# Autodesk Inventor assembly: 00_Linear_Stage_NEMA11_china
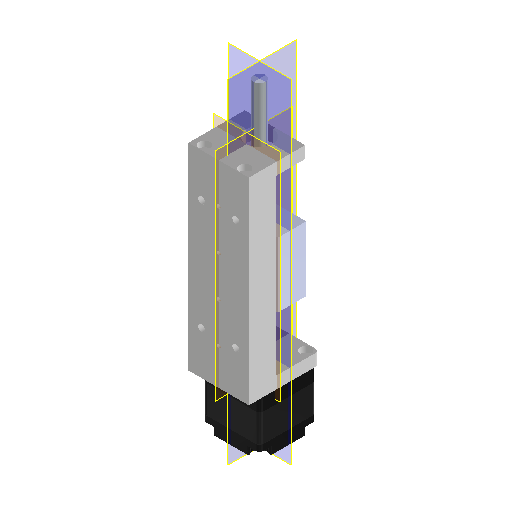
[picture p0: Inventor's stored thumbnail of the model, 512x512]
Saved by Autodesk Inventor 2023 (Build 270158000, 158)
## iProperties
Created: 2022-01-12
Part Number: 00_Linear_Stage_NEMA11_china
Document SubType Name: Assembly
Designer: diederichbenedict
Sending System: Autodesk Inventor 2022
Preprocessor: ST-DEVELOPER v18.1
Title: C:\Users\diederichbenedict\Dropbox\Dokumente\Promotion\PROJECTS\UC2\02_CAD\INVENTOR\uc2_v3\00_Linear_Stage_NEMA11_china.stp
Author: diederichbenedict
## Documents named in this file (6)
- C:\Users\diederichbenedict\Downloads\UC2 setup design\UC2 setup design\00_Linear_Stage_NEMA11_china.iam
- C:\Users\diederichbenedict\Downloads\UC2 setup design\UC2 setup design\Actuator_MGN9.ipt
- C:\Users\diederichbenedict\Downloads\UC2 setup design\UC2 setup design\Actuator_MGN9C.ipt
- C:\Users\diederichbenedict\Downloads\UC2 setup design\UC2 setup design\Actuator_movable.ipt
- C:\Users\diederichbenedict\Downloads\UC2 setup design\UC2 setup design\00_Carriage.ipt
- C:\Users\diederichbenedict\Downloads\UC2 setup design\UC2 setup design\00_NEMA11_spindle.ipt
## Components (5 placed, 5 different names)
1. Actuator_MGN9:1 — Passend:6
2. Actuator_MGN9C:1 — Passend:6, Passend:7
3. 00_Carriage:1 — Fluchtend:1, Fluchtend:2
4. 00_NEMA11_spindle:1 — Passend:4, Winkel:2, Passend:5
5. Actuator_movable — Fluchtend:1, Fluchtend:2, Passend:4, Winkel:2, Passend:5, Passend:7
## Relationships (11: Mate 7, Angle 2, Flush 2)
- [Mate]: 00_Carriage:1 ↔ 00_NEMA11_spindle:1
- [Mate]: 00_NEMA11_spindle:1 ↔ Actuator_movable
- [Mate]: 00_NEMA11_spindle:1 ↔ Actuator_movable
- [Angle] (0 deg): 00_Carriage:1 ↔ Actuator_movable
- Fluchtend:1 [Flush]: 00_Carriage:1 ↔ Actuator_movable
- Fluchtend:2 [Flush] (-14.9 mm): 00_Carriage:1 ↔ Actuator_movable
- Passend:4 [Mate]: 00_NEMA11_spindle:1 ↔ Actuator_movable
- Winkel:2 [Angle] (0 deg): 00_NEMA11_spindle:1 ↔ Actuator_movable
- Passend:5 [Mate]: 00_NEMA11_spindle:1 ↔ Actuator_movable
- Passend:6 [Mate]: Actuator_MGN9:1 ↔ Actuator_MGN9C:1
- Passend:7 [Mate]: Actuator_MGN9C:1 ↔ Actuator_movable
